# Autodesk Inventor assembly: L12
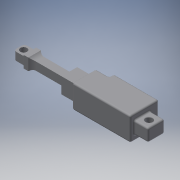
[picture p0: Inventor's stored thumbnail of the model, 180x180]
Saved by Autodesk Inventor 2016 (Build 200138000, 138)
## iProperties
Created: 2015-10-13
Part Number: L12
Document SubType Name: Assembly
Designer: eedoga
Author: eedoga
## Documents named in this file (4)
- C:\Users\master\Documents\!ActiveArm\L12.iam
- C:\Users\master\Documents\!ActiveArm\base.ipt
- C:\Users\master\Documents\!ActiveArm\arm-seg1.ipt
- C:\Users\master\Documents\!ActiveArm\arm-seg2.ipt
## Components (3 placed, 3 different names)
1. base:1
2. arm-seg1:1 — Mate:1
3. arm-seg2:1 — Mate:1
## Relationships (1: Mate 1)
- Mate:1: arm-seg1:1 ↔ arm-seg2:1
